# Autodesk Inventor assembly: Full Pin
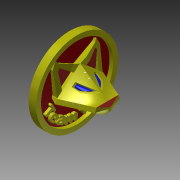
[picture p0: Inventor's stored thumbnail of the model, 180x180]
Saved by Autodesk Inventor 2014 (Build 180170000, 170)
## iProperties
Created: 2015-01-18
Part Number: Full Pin
Document SubType Name: Assembly
Designer: Spooner
Author: Spooner
## Documents named in this file (6)
- C:\Users\Spooner\Documents\Inventor\RoboCat Gen 2\Full Pin.iam
- C:\Users\Spooner\Documents\Inventor\RoboCat Gen 2\roboCat-Pin 2015, Yellow.ipt
- C:\Users\Spooner\Documents\Inventor\RoboCat Gen 2\Bakground.ipt
- C:\Users\Spooner\Documents\Inventor\RoboCat Gen 2\Ears.ipt
- C:\Users\Spooner\Documents\Inventor\RoboCat Gen 2\Eyes.ipt
- C:\Users\Spooner\Documents\Inventor\RoboCat Gen 2\Nose.ipt
## Components (5 placed, 5 different names)
1. roboCat-Pin 2015, Yellow:1 — Mate:1, Mate:2, Mate:3, Mate:4, Mate:5, Mate:6, Mate:7, Mate:8, Mate:9, Mate:10, Mate:11, Angle:2, Insert:1, Angle:3
2. Bakground:1 — Insert:1, Angle:3
3. Ears:1 — Mate:4, Mate:5, Mate:6
4. Eyes:1 — Mate:1, Mate:2, Mate:3
5. Nose:1 — Mate:7, Mate:8, Mate:9
## Relationships (15: Mate 12, Angle 2, Insert 1)
- Mate:1: roboCat-Pin 2015, Yellow:1 ↔ Eyes:1
- Mate:2: roboCat-Pin 2015, Yellow:1 ↔ Eyes:1
- Mate:3: roboCat-Pin 2015, Yellow:1 ↔ Eyes:1
- Mate:4: roboCat-Pin 2015, Yellow:1 ↔ Ears:1
- Mate:5: roboCat-Pin 2015, Yellow:1 ↔ Ears:1
- Mate:6: roboCat-Pin 2015, Yellow:1 ↔ Ears:1
- Mate:7: roboCat-Pin 2015, Yellow:1 ↔ Nose:1
- Mate:8: roboCat-Pin 2015, Yellow:1 ↔ Nose:1
- Mate:9: roboCat-Pin 2015, Yellow:1 ↔ Nose:1
- Mate:10: roboCat-Pin 2015, Yellow:1
- Mate:11: roboCat-Pin 2015, Yellow:1
- Mate:12
- Angle:2 (270 deg): roboCat-Pin 2015, Yellow:1
- Insert:1: roboCat-Pin 2015, Yellow:1 ↔ Bakground:1
- Angle:3 (180 deg): roboCat-Pin 2015, Yellow:1 ↔ Bakground:1
